# Autodesk Inventor assembly: main assembly
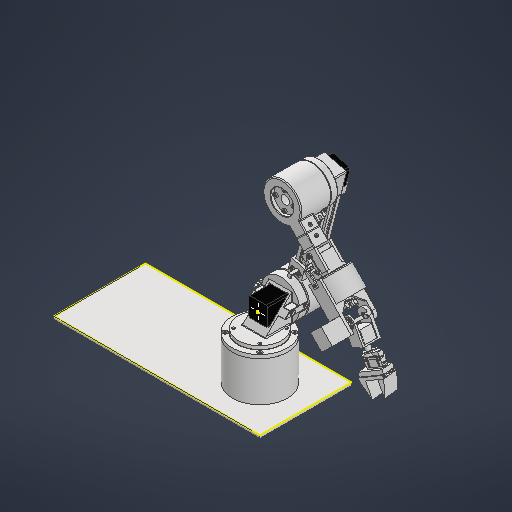
[picture p0: Inventor's stored thumbnail of the model, 512x512]
Saved by Autodesk Inventor 2026.1 (Build 301233020, 233B)
## iProperties
Created: 2025-07-04
Part Number: main assembly
Document SubType Name: Assembly
Designer: gavin
Author: gavin
## Documents named in this file (41)
- F:\temp data disk\Github\6-DOF-Robot-Arm\3D-model\robot armT 2(CAD file)\main assembly.iam
- F:\temp data disk\Github\6-DOF-Robot-Arm\3D-model\robot armT 2(CAD file)\stepper 42x48 - 27.ipt
- F:\temp data disk\Github\6-DOF-Robot-Arm\3D-model\robot armT 2(CAD file)\28stepper27.ipt
- F:\temp data disk\Github\6-DOF-Robot-Arm\3D-model\robot armT 2(CAD file)\CSN 02 4630 - 6009.ipt
- F:\temp data disk\Github\6-DOF-Robot-Arm\3D-model\robot armT 2(CAD file)\CNS 2862 B2116 - 6007 - 35 x 62 x 14.ipt
- F:\temp data disk\Github\6-DOF-Robot-Arm\3D-model\robot armT 2(CAD file)\base plate.ipt
- F:\temp data disk\Github\6-DOF-Robot-Arm\3D-model\robot armT 2(CAD file)\stepper 42x60 -50 .ipt
- F:\temp data disk\Github\6-DOF-Robot-Arm\3D-model\robot armT 2(CAD file)\j2 42 motor mount.ipt
- F:\temp data disk\Github\6-DOF-Robot-Arm\3D-model\robot armT 2(CAD file)\j1 assmble.iam
- F:\temp data disk\Github\6-DOF-Robot-Arm\3D-model\robot armT 2(CAD file)\optic endstop module.ipt
- F:\temp data disk\Github\6-DOF-Robot-Arm\3D-model\robot armT 2(CAD file)\j2j3 alumi ext.ipt
- F:\temp data disk\Github\6-DOF-Robot-Arm\3D-model\robot armT 2(CAD file)\j3 motor mount.ipt
- F:\temp data disk\Github\6-DOF-Robot-Arm\3D-model\robot armT 2(CAD file)\j3j4 alumi ext.ipt
- F:\temp data disk\Github\6-DOF-Robot-Arm\3D-model\robot armT 2(CAD file)\j2 endstop blocker.ipt
- F:\temp data disk\Github\6-DOF-Robot-Arm\3D-model\robot armT 2(CAD file)\j3 endstop blocker.ipt
- F:\temp data disk\Github\6-DOF-Robot-Arm\3D-model\robot armT 2(CAD file)\6mm axle hub.ipt
- F:\temp data disk\Github\6-DOF-Robot-Arm\3D-model\robot armT 2(CAD file)\j4 motor mount.ipt
- F:\temp data disk\Github\6-DOF-Robot-Arm\3D-model\robot armT 2(CAD file)\j4 motor mount cover.ipt
- F:\temp data disk\Github\6-DOF-Robot-Arm\3D-model\robot armT 2(CAD file)\j4 moving part.ipt
- F:\temp data disk\Github\6-DOF-Robot-Arm\3D-model\robot armT 2(CAD file)\nema 11x25.ipt
- F:\temp data disk\Github\6-DOF-Robot-Arm\3D-model\robot armT 2(CAD file)\5mm axle hub.ipt
- F:\temp data disk\Github\6-DOF-Robot-Arm\3D-model\robot armT 2(CAD file)\bearing 22-M6.ipt
- F:\temp data disk\Github\6-DOF-Robot-Arm\3D-model\robot armT 2(CAD file)\j6 motor mount v2.ipt
- F:\temp data disk\Github\6-DOF-Robot-Arm\3D-model\robot armT 2(CAD file)\j4 endstop blocker.ipt
- F:\temp data disk\Github\6-DOF-Robot-Arm\3D-model\robot armT 2(CAD file)\sg90 long claw.iam
- F:\temp data disk\Github\6-DOF-Robot-Arm\3D-model\robot armT 2(CAD file)\35x40 stepper.ipt
- F:\temp data disk\Github\6-DOF-Robot-Arm\3D-model\robot armT 2(CAD file)\j3 moving part option3.ipt
- F:\temp data disk\Github\6-DOF-Robot-Arm\3D-model\robot armT 2(CAD file)\z21 8x18.ipt
- F:\temp data disk\Github\6-DOF-Robot-Arm\3D-model\robot armT 2(CAD file)\18mm hub.ipt
- F:\temp data disk\Github\6-DOF-Robot-Arm\3D-model\robot armT 2(CAD file)\j2 moving part option2.ipt
- F:\temp data disk\Github\6-DOF-Robot-Arm\3D-model\robot armT 2(CAD file)\M5 heat set inserts.ipt
- F:\temp data disk\Github\6-DOF-Robot-Arm\3D-model\robot armT 2(CAD file)\AS 1427 - M3 x 6(5) II.ipt
- F:\temp data disk\Github\6-DOF-Robot-Arm\3D-model\robot armT 2(CAD file)\M3 heat set insert.ipt
- C:\Users\gavin\Documents\Inventor\Content Center Files\R2026\en-US\CNS 4557\CNS 4557 - M5 x 0.8 x 12.ipt
- F:\temp data disk\Github\6-DOF-Robot-Arm\3D-model\robot armT 2(CAD file)\CNS 4557 - M4 x 0.7 x 10.ipt
- F:\temp data disk\Github\6-DOF-Robot-Arm\3D-model\robot armT 2(CAD file)\AS 1474 - M4(1).ipt
- F:\temp data disk\Github\6-DOF-Robot-Arm\3D-model\robot armT 2(CAD file)\AS 1474 - M3(1).ipt
- C:\Users\gavin\Documents\Inventor\Content Center Files\R2026\en-US\AS 1112 (4)\AS 1112 - M6(2).ipt
- C:\Users\gavin\Documents\Inventor\Content Center Files\R2026\en-US\ASME ANSI B18.3.5M(2)\ASME_ANSI B18.3.5M - M3x6(2).ipt
- C:\Users\gavin\Documents\Inventor\Content Center Files\R2026\en-US\CNS 3932\CNS 3932 - M 4 x 0.7 x 10.ipt
- C:\Users\gavin\Documents\Inventor\Content Center Files\R2026\en-US\IS 7483\IS 7483 - M3 x 14.ipt
## Components (130 placed, 40 different names)
1. base plate:1 — Flush:5
2. j1 assmble:1 [sub-assembly]
3. stepper 42x48 - 27:2 — Mate:45, Mate:46, Mate:47, Mate:110, Flush:18
4. CSN 02 4630 - 6009:1 — Mate:48, Mate:49, Rotational:15
5. CSN 02 4630 - 6009:2 — Mate:16, Mate:29
6. CNS 2862 B2116 - 6007 - 35 x 62 x 14:1 — Mate:63, Mate:64, Rotational:16
7. stepper 42x60 -50 :1 — Mate:16, Mate:27, Mate:28, Mate:113, Flush:20
8. j2 42 motor mount:1 — Mate:27, Mate:28, Mate:29, Mate:33, Mate:34, Mate:35, Rigid:12, Rigid:13, Rigid:99, Rigid:100, Rigid:101, Rigid:102
9. optic endstop module:1 — Mate:33, Mate:34, Mate:35, Flush:10, Rigid:10, Rigid:11
10. j2j3 alumi ext:1 — Rigid:5, Rigid:7
11. j2j3 alumi ext:2 — Rigid:6
12. j3 motor mount:1 — Mate:45, Mate:46, Mate:47, Mate:48, Mate:49, Flush:11, Flush:12, Mate:59, Rigid:7, Mate:132, Rigid:65, Rigid:66, Rigid:67, Rigid:68, Rigid:95, Rigid:96, Rigid:97, Rigid:98
13. j3j4 alumi ext:1 — Rigid:4, Rigid:8
14. optic endstop module:2 — Mate:129, Mate:130, Mate:131, Rigid:20, Rigid:21, Rigid:22, Rigid:23
15. j2 endstop blocker:1 — Flush:10, Mate:117, Mate:118, Mate:119, Rigid:14, Rigid:15, Rigid:16, Rigid:17
16. j3 endstop blocker:1 — Flush:11, Flush:12, Mate:59, Mate:132, Rigid:18, Rigid:19, Rigid:24, Rigid:25
17. 6mm axle hub:1 — Mate:123, Mate:124, Mate:125
18. j4 motor mount:1 — Flush:14, Flush:15, Mate:62, Mate:63, Mate:65, Mate:71, Mate:72, Mate:73, Flush:21, Rigid:8, Rigid:9, Rigid:27, Rigid:28, Rigid:72, Rigid:75
19. j4 motor mount cover:1 — Flush:14, Flush:15, Mate:62, Mate:64, Mate:65
20. 28stepper27:1 — Rigid:9
21. optic endstop module:3 — Mate:71, Mate:72, Mate:73, Rigid:29, Rigid:30
22. j4 moving part:1 — Mate:74, Mate:76, Mate:86, Mate:87, Mate:104, Mate:105, Mate:107, Mate:108, Mate:109, Mate:123, Mate:124, Mate:125, Rotational:16, Mate:126, Mate:127, Rigid:26, Rigid:32, Rigid:33, Rigid:76, Rigid:77, Rigid:78, Rigid:79, Rigid:89, Rigid:90
23. nema 11x25:1 — Mate:88, Mate:89, Mate:102, Mate:103, Mate:128
24. optic endstop module:4 — Mate:74, Mate:76, Mate:107, Rigid:34, Rigid:35
25. 5mm axle hub:1 — Rigid:1, Rotational:12
26. bearing 22-M6:1 — Mate:86, Mate:87
27. j6 motor mount v2:1 — Mate:88, Mate:89, Rotational:12, Mate:128, Rigid:80, Rigid:81, Rigid:82, Rigid:83, Rigid:88
28. j4 endstop blocker:1 — Mate:108, Mate:109, Mate:126, Rigid:31
29. sg90 long claw:1 [sub-assembly] — Mate:99, Mate:100, Mate:101, Mate:103, Rigid:91, Rigid:92, Rigid:93, Rigid:94
30. 5mm axle hub:2 — Mate:99, Mate:100, Mate:101, Mate:102
31. 35x40 stepper:1 — Mate:104, Mate:105, Rigid:1, Mate:127
32. j3 moving part option3:1 — Rigid:4, Mate:120, Mate:121, Mate:122, Rotational:15, Flush:21, Mate:129, Mate:130, Mate:131, Rigid:40, Rigid:41, Rigid:42, Rigid:43, Rigid:73, Rigid:74
33. z21 8x18:1 — Mate:110, Flush:18
34. 18mm hub:1 — Mate:120, Mate:121, Mate:122, Rigid:44, Rigid:45, Rigid:46, Rigid:47
35. j2 moving part option2:1 — Rigid:5, Mate:114, Mate:115, Mate:116, Mate:117, Mate:118, Mate:119, Rigid:6, Rigid:36, Rigid:37, Rigid:38, Rigid:39, Rigid:59, Rigid:60, Rigid:61, Rigid:62
36. z21 8x18:2 — Rotational:14, Mate:113, Flush:20
37. 18mm hub:2 — Rotational:14, Mate:114, Mate:115, Mate:116, Rigid:48, Rigid:49, Rigid:50, Rigid:51
38. AS 1427 - M3 x 6(5) II:1 — Rigid:16
39. AS 1427 - M3 x 6(5) II:2 — Rigid:23
40. AS 1427 - M3 x 6(5) II:3 — Rigid:24
41. AS 1427 - M3 x 6(5) II:4 — Rigid:22
42. AS 1427 - M3 x 6(5) II:5 — Rigid:17
43. AS 1427 - M3 x 6(5) II:6 — Rigid:25
44. AS 1427 - M3 x 6(5) II:7 — Rigid:10
45. AS 1427 - M3 x 6(5) II:8 — Rigid:11
46. M3 heat set insert:1 — Rigid:15
47. M3 heat set insert:2 — Rigid:13
48. M3 heat set insert:3 — Rigid:26
49. M3 heat set insert:4 — Rigid:32
50. M3 heat set insert:5 — Rigid:28
51. M3 heat set insert:6 — Rigid:19
52. M3 heat set insert:7 — Rigid:20
53. M3 heat set insert:8 — Rigid:12
54. M3 heat set insert:9 — Rigid:14
55. M3 heat set insert:10 — Rigid:33
56. M3 heat set insert:14 — Rigid:27
57. M3 heat set insert:15 — Rigid:18
58. M3 heat set insert:18 — Rigid:21
59. AS 1427 - M3 x 6(5) II:9 — Rigid:29
60. AS 1427 - M3 x 6(5) II:10 — Rigid:35
61. AS 1427 - M3 x 6(5) II:11 — Rigid:31
62. AS 1427 - M3 x 6(5) II:12 — Rigid:30
63. AS 1427 - M3 x 6(5) II:13 — Rigid:34
64. M5 heat set inserts:5 — Rigid:39
65. M5 heat set inserts:6 — Rigid:36
66. M5 heat set inserts:10 — Rigid:42
67. M5 heat set inserts:11 — Rigid:41
68. M5 heat set inserts:12 — Rigid:40
69. M5 heat set inserts:13 — Rigid:38
70. M5 heat set inserts:14 — Rigid:37
71. M5 heat set inserts:18 — Rigid:43
72. CNS 4557 M5 x 12:1 — Rigid:45
73. CNS 4557 M5 x 12:2 — Rigid:44
74. CNS 4557 M5 x 12:3 — Rigid:49
75. CNS 4557 M5 x 12:4 — Rigid:48
76. CNS 4557 M5 x 12:5 — Rigid:47
77. CNS 4557 M5 x 12:6 — Rigid:46
78. CNS 4557 M5 x 12:7 — Rigid:51
79. CNS 4557 M5 x 12:8 — Rigid:50
80. CNS 4557 - M4 x 0.7 x 10:1 — Rigid:64, Rigid:65
81. CNS 4557 - M4 x 0.7 x 10:2 — Rigid:57, Rigid:60
82. CNS 4557 - M4 x 0.7 x 10:3 — Rigid:55, Rigid:74
83. CNS 4557 - M4 x 0.7 x 10:4 — Rigid:53, Rigid:67
84. CNS 4557 - M4 x 0.7 x 10:5 — Rigid:58, Rigid:59
85. CNS 4557 - M4 x 0.7 x 10:6 — Rigid:56, Rigid:62
86. CNS 4557 - M4 x 0.7 x 10:7 — Rigid:54, Rigid:68
87. CNS 4557 - M4 x 0.7 x 10:8 — Rigid:52, Rigid:61
88. CNS 4557 - M4 x 0.7 x 10:9 — Rigid:71, Rigid:72
89. CNS 4557 - M4 x 0.7 x 10:10 — Rigid:70, Rigid:73
90. CNS 4557 - M4 x 0.7 x 10:11 — Rigid:63, Rigid:66
91. CNS 4557 - M4 x 0.7 x 10:12 — Rigid:69, Rigid:75
92. AS 1474 - M4(1):1 — Rigid:57
93. AS 1474 - M4(1):2 — Rigid:55
94. AS 1474 - M4(1):3 — Rigid:92
95. AS 1474 - M4(1):4 — Rigid:91
96. AS 1474 - M4(1):5 — Rigid:56
97. AS 1474 - M4(1):6 — Rigid:53
98. AS 1474 - M4(1):7 — Rigid:54
99. AS 1474 - M4(1):11 — Rigid:64
100. AS 1474 - M4(1):12 — Rigid:63
101. AS 1474 - M4(1):13 — Rigid:71
102. AS 1474 - M4(1):14 — Rigid:69
103. AS 1474 - M4(1):15 — Rigid:70
104. AS 1474 - M4(1):16 — Rigid:52
105. AS 1474 - M4(1):18 — Rigid:58
106. AS 1474 - M3(1):1 — Rigid:87
107. AS 1474 - M3(1):2 — Rigid:86
108. AS 1474 - M3(1):3 — Rigid:84
109. AS 1474 - M3(1):5 — Rigid:85
110. AS 1112 (4) - Metric M6:1 — Rigid:88
111. Broached Hexagon Socket Flat Countersunk Head Cap Screws - Metric M3x6:1 — Rigid:77
112. Broached Hexagon Socket Flat Countersunk Head Cap Screws - Metric M3x6:2 — Rigid:78
113. Broached Hexagon Socket Flat Countersunk Head Cap Screws - Metric M3x6:3 — Rigid:80, Rigid:84
114. Broached Hexagon Socket Flat Countersunk Head Cap Screws - Metric M3x6:4 — Rigid:81, Rigid:85
115. Broached Hexagon Socket Flat Countersunk Head Cap Screws - Metric M3x6:5 — Rigid:76
116. Broached Hexagon Socket Flat Countersunk Head Cap Screws - Metric M3x6:6 — Rigid:79
117. CNS 3932 M 4 x 10:1 — Rigid:89
118. CNS 3932 M 4 x 10:4 — Rigid:90
119. IS 7483 M3 x 14:1 — Rigid:93
120. IS 7483 M3 x 14:2 — Rigid:94
121. Broached Hexagon Socket Flat Countersunk Head Cap Screws - Metric M3x6:7 — Rigid:83, Rigid:87
122. Broached Hexagon Socket Flat Countersunk Head Cap Screws - Metric M3x6:8 — Rigid:82, Rigid:86
123. Broached Hexagon Socket Flat Countersunk Head Cap Screws - Metric M3x6:9 — Rigid:97
124. Broached Hexagon Socket Flat Countersunk Head Cap Screws - Metric M3x6:10 — Rigid:95
125. Broached Hexagon Socket Flat Countersunk Head Cap Screws - Metric M3x6:11 — Rigid:99
126. Broached Hexagon Socket Flat Countersunk Head Cap Screws - Metric M3x6:12 — Rigid:101
127. Broached Hexagon Socket Flat Countersunk Head Cap Screws - Metric M3x6:13 — Rigid:96
128. Broached Hexagon Socket Flat Countersunk Head Cap Screws - Metric M3x6:14 — Rigid:98
129. Broached Hexagon Socket Flat Countersunk Head Cap Screws - Metric M3x6:15 — Rigid:100
130. Broached Hexagon Socket Flat Countersunk Head Cap Screws - Metric M3x6:16 — Rigid:102
## Relationships (184: WeldJoint 100, Mate 64, Flush 10, RevoluteJoint 10)
- [Mate]: j1 assmble:1
- [Flush]: base plate:1 ↔ j1 assmble:1
- [Mate]: base plate:1 ↔ j1 assmble:1
- Flush:5: base plate:1
- Mate:16: CSN 02 4630 - 6009:2 ↔ stepper 42x60 -50 :1
- [Mate] (20 mm): j1 assmble:1 ↔ stepper 42x60 -50 :1
- [Mate]: j1 assmble:1 ↔ j2 42 motor mount:1
- [Mate]: base plate:1 ↔ j1 assmble:1
- [Mate]: j1 assmble:1 ↔ j2 42 motor mount:1
- [Mate]: j1 assmble:1 ↔ j2 42 motor mount:1
- Mate:27: stepper 42x60 -50 :1 ↔ j2 42 motor mount:1
- Mate:28: stepper 42x60 -50 :1 ↔ j2 42 motor mount:1
- Mate:29: CSN 02 4630 - 6009:2 ↔ j2 42 motor mount:1
- [RevoluteJoint]: base plate:1 ↔ j1 assmble:1
- [RevoluteJoint]: base plate:1 ↔ j1 assmble:1
- [RevoluteJoint]: base plate:1 ↔ j1 assmble:1
- [RevoluteJoint]: base plate:1 ↔ j1 assmble:1
- [RevoluteJoint]: base plate:1 ↔ j1 assmble:1
- [RevoluteJoint]: base plate:1 ↔ j1 assmble:1
- Mate:33: j2 42 motor mount:1 ↔ optic endstop module:1
- Mate:34: j2 42 motor mount:1 ↔ optic endstop module:1
- Mate:35: j2 42 motor mount:1 ↔ optic endstop module:1
- Mate:45: stepper 42x48 - 27:2 ↔ j3 motor mount:1
- Mate:46 (0.075 mm): stepper 42x48 - 27:2 ↔ j3 motor mount:1
- Mate:47: stepper 42x48 - 27:2 ↔ j3 motor mount:1
- Mate:48: CSN 02 4630 - 6009:1 ↔ j3 motor mount:1
- Mate:49: CSN 02 4630 - 6009:1 ↔ j3 motor mount:1
- Flush:10: optic endstop module:1 ↔ j2 endstop blocker:1
- Flush:11: j3 motor mount:1 ↔ j3 endstop blocker:1
- Flush:12: j3 motor mount:1 ↔ j3 endstop blocker:1
- Flush:14: j4 motor mount:1 ↔ j4 motor mount cover:1
- Flush:15: j4 motor mount:1 ↔ j4 motor mount cover:1
- Mate:59: j3 motor mount:1 ↔ j3 endstop blocker:1
- Mate:62: j4 motor mount:1 ↔ j4 motor mount cover:1
- Mate:63: CNS 2862 B2116 - 6007 - 35 x 62 x 14:1 ↔ j4 motor mount:1
- Mate:64: CNS 2862 B2116 - 6007 - 35 x 62 x 14:1 ↔ j4 motor mount cover:1
- Mate:65: j4 motor mount:1 ↔ j4 motor mount cover:1
- Mate:71: j4 motor mount:1 ↔ optic endstop module:3
- Mate:72: j4 motor mount:1 ↔ optic endstop module:3
- Mate:73: j4 motor mount:1 ↔ optic endstop module:3
- Mate:74: j4 moving part:1 ↔ optic endstop module:4
- Mate:76: j4 moving part:1 ↔ optic endstop module:4
- Mate:86: j4 moving part:1 ↔ bearing 22-M6:1
- Mate:87: j4 moving part:1 ↔ bearing 22-M6:1
- Mate:88: nema 11x25:1 ↔ j6 motor mount v2:1
- Mate:89: nema 11x25:1 ↔ j6 motor mount v2:1
- Mate:99: sg90 long claw:1 ↔ 5mm axle hub:2
- Mate:100: sg90 long claw:1 ↔ 5mm axle hub:2
- Mate:101: sg90 long claw:1 ↔ 5mm axle hub:2
- Mate:102: nema 11x25:1 ↔ 5mm axle hub:2
- Mate:103: nema 11x25:1 ↔ sg90 long claw:1
- Mate:104: j4 moving part:1 ↔ 35x40 stepper:1
- Mate:105: j4 moving part:1 ↔ 35x40 stepper:1
- Rigid:1 [WeldJoint]: 5mm axle hub:1 ↔ 35x40 stepper:1
- Rotational:12 [RevoluteJoint]: 5mm axle hub:1 ↔ j6 motor mount v2:1
- Mate:107: j4 moving part:1 ↔ optic endstop module:4
- Mate:108: j4 moving part:1 ↔ j4 endstop blocker:1
- Mate:109: j4 moving part:1 ↔ j4 endstop blocker:1
- Mate:110: stepper 42x48 - 27:2 ↔ z21 8x18:1
- Flush:18: stepper 42x48 - 27:2 ↔ z21 8x18:1
- Rotational:14 [RevoluteJoint] (-3.71 mm): z21 8x18:2 ↔ 18mm hub:2
- Mate:113: stepper 42x60 -50 :1 ↔ z21 8x18:2
- Flush:20: stepper 42x60 -50 :1 ↔ z21 8x18:2
- Rigid:4 [WeldJoint]: j3j4 alumi ext:1 ↔ j3 moving part option3:1
- Rigid:5 [WeldJoint]: j2j3 alumi ext:1 ↔ j2 moving part option2:1
- Mate:114: j2 moving part option2:1 ↔ 18mm hub:2
- Mate:115: j2 moving part option2:1 ↔ 18mm hub:2
- Mate:116: j2 moving part option2:1 ↔ 18mm hub:2
- Mate:117: j2 endstop blocker:1 ↔ j2 moving part option2:1
- Mate:118: j2 endstop blocker:1 ↔ j2 moving part option2:1
- Mate:119: j2 endstop blocker:1 ↔ j2 moving part option2:1
- Rigid:6 [WeldJoint]: j2j3 alumi ext:2 ↔ j2 moving part option2:1
- Rigid:7 [WeldJoint]: j2j3 alumi ext:1 ↔ j3 motor mount:1
- Mate:120: j3 moving part option3:1 ↔ 18mm hub:1
- Mate:121: j3 moving part option3:1 ↔ 18mm hub:1
- Mate:122: j3 moving part option3:1 ↔ 18mm hub:1
- Rotational:15 [RevoluteJoint]: CSN 02 4630 - 6009:1 ↔ j3 moving part option3:1
- Flush:21: j4 motor mount:1 ↔ j3 moving part option3:1
- Rigid:8 [WeldJoint]: j3j4 alumi ext:1 ↔ j4 motor mount:1
- Rigid:9 [WeldJoint]: j4 motor mount:1 ↔ 28stepper27:1
- Mate:123: 6mm axle hub:1 ↔ j4 moving part:1
- Mate:124: 6mm axle hub:1 ↔ j4 moving part:1
- Mate:125: 6mm axle hub:1 ↔ j4 moving part:1
- Rotational:16 [RevoluteJoint]: CNS 2862 B2116 - 6007 - 35 x 62 x 14:1 ↔ j4 moving part:1
- Mate:126: j4 moving part:1 ↔ j4 endstop blocker:1
- Mate:127: j4 moving part:1 ↔ 35x40 stepper:1
- Mate:128: nema 11x25:1 ↔ j6 motor mount v2:1
- Mate:129: optic endstop module:2 ↔ j3 moving part option3:1
- Mate:130: optic endstop module:2 ↔ j3 moving part option3:1
- Mate:131: optic endstop module:2 ↔ j3 moving part option3:1
- Mate:132: j3 motor mount:1 ↔ j3 endstop blocker:1
- Rigid:10 [WeldJoint]: optic endstop module:1 ↔ AS 1427 - M3 x 6(5) II:7
- Rigid:11 [WeldJoint]: optic endstop module:1 ↔ AS 1427 - M3 x 6(5) II:8
- Rigid:12 [WeldJoint]: j2 42 motor mount:1 ↔ M3 heat set insert:8
- Rigid:13 [WeldJoint]: j2 42 motor mount:1 ↔ M3 heat set insert:2
- Rigid:14 [WeldJoint]: j2 endstop blocker:1 ↔ M3 heat set insert:9
- Rigid:15 [WeldJoint]: j2 endstop blocker:1 ↔ M3 heat set insert:1
- Rigid:16 [WeldJoint]: j2 endstop blocker:1 ↔ AS 1427 - M3 x 6(5) II:1
- Rigid:17 [WeldJoint]: j2 endstop blocker:1 ↔ AS 1427 - M3 x 6(5) II:5
- Rigid:18 [WeldJoint]: j3 endstop blocker:1 ↔ M3 heat set insert:15
- Rigid:19 [WeldJoint]: j3 endstop blocker:1 ↔ M3 heat set insert:6
- Rigid:20 [WeldJoint]: optic endstop module:2 ↔ M3 heat set insert:7
- Rigid:21 [WeldJoint]: optic endstop module:2 ↔ M3 heat set insert:18
- Rigid:22 [WeldJoint]: optic endstop module:2 ↔ AS 1427 - M3 x 6(5) II:4
- Rigid:23 [WeldJoint]: optic endstop module:2 ↔ AS 1427 - M3 x 6(5) II:2
- Rigid:24 [WeldJoint]: j3 endstop blocker:1 ↔ AS 1427 - M3 x 6(5) II:3
- Rigid:25 [WeldJoint]: j3 endstop blocker:1 ↔ AS 1427 - M3 x 6(5) II:6
- Rigid:26 [WeldJoint]: j4 moving part:1 ↔ M3 heat set insert:3
- Rigid:27 [WeldJoint]: j4 motor mount:1 ↔ M3 heat set insert:14
- Rigid:28 [WeldJoint]: j4 motor mount:1 ↔ M3 heat set insert:5
- Rigid:29 [WeldJoint]: optic endstop module:3 ↔ AS 1427 - M3 x 6(5) II:9
- Rigid:30 [WeldJoint]: optic endstop module:3 ↔ AS 1427 - M3 x 6(5) II:12
- Rigid:31 [WeldJoint]: j4 endstop blocker:1 ↔ AS 1427 - M3 x 6(5) II:11
- Rigid:32 [WeldJoint]: j4 moving part:1 ↔ M3 heat set insert:4
- Rigid:33 [WeldJoint]: j4 moving part:1 ↔ M3 heat set insert:10
- Rigid:34 [WeldJoint]: optic endstop module:4 ↔ AS 1427 - M3 x 6(5) II:13
- Rigid:35 [WeldJoint]: optic endstop module:4 ↔ AS 1427 - M3 x 6(5) II:10
- Rigid:36 [WeldJoint]: j2 moving part option2:1 ↔ M5 heat set inserts:6
- Rigid:37 [WeldJoint]: j2 moving part option2:1 ↔ M5 heat set inserts:14
- Rigid:38 [WeldJoint]: j2 moving part option2:1 ↔ M5 heat set inserts:13
- Rigid:39 [WeldJoint]: j2 moving part option2:1 ↔ M5 heat set inserts:5
- Rigid:40 [WeldJoint]: j3 moving part option3:1 ↔ M5 heat set inserts:12
- Rigid:41 [WeldJoint]: j3 moving part option3:1 ↔ M5 heat set inserts:11
- Rigid:42 [WeldJoint]: j3 moving part option3:1 ↔ M5 heat set inserts:10
- Rigid:43 [WeldJoint]: j3 moving part option3:1 ↔ M5 heat set inserts:18
- Rigid:44 [WeldJoint]: 18mm hub:1 ↔ CNS 4557 M5 x 12:2
- Rigid:45 [WeldJoint]: 18mm hub:1 ↔ CNS 4557 M5 x 12:1
- Rigid:46 [WeldJoint]: 18mm hub:1 ↔ CNS 4557 M5 x 12:6
- Rigid:47 [WeldJoint]: 18mm hub:1 ↔ CNS 4557 M5 x 12:5
- Rigid:48 [WeldJoint]: 18mm hub:2 ↔ CNS 4557 M5 x 12:4
- Rigid:49 [WeldJoint]: 18mm hub:2 ↔ CNS 4557 M5 x 12:3
- Rigid:50 [WeldJoint]: 18mm hub:2 ↔ CNS 4557 M5 x 12:8
- Rigid:51 [WeldJoint]: 18mm hub:2 ↔ CNS 4557 M5 x 12:7
- Rigid:52 [WeldJoint] (10 mm): CNS 4557 - M4 x 0.7 x 10:8 ↔ AS 1474 - M4(1):16
- Rigid:53 [WeldJoint]: CNS 4557 - M4 x 0.7 x 10:4 ↔ AS 1474 - M4(1):6
- Rigid:54 [WeldJoint]: CNS 4557 - M4 x 0.7 x 10:7 ↔ AS 1474 - M4(1):7
- Rigid:55 [WeldJoint]: CNS 4557 - M4 x 0.7 x 10:3 ↔ AS 1474 - M4(1):2
- Rigid:56 [WeldJoint]: CNS 4557 - M4 x 0.7 x 10:6 ↔ AS 1474 - M4(1):5
- Rigid:57 [WeldJoint]: CNS 4557 - M4 x 0.7 x 10:2 ↔ AS 1474 - M4(1):1
- Rigid:58 [WeldJoint]: CNS 4557 - M4 x 0.7 x 10:5 ↔ AS 1474 - M4(1):18
- Rigid:59 [WeldJoint]: j2 moving part option2:1 ↔ CNS 4557 - M4 x 0.7 x 10:5
- Rigid:60 [WeldJoint]: j2 moving part option2:1 ↔ CNS 4557 - M4 x 0.7 x 10:2
- Rigid:61 [WeldJoint]: j2 moving part option2:1 ↔ CNS 4557 - M4 x 0.7 x 10:8
- Rigid:62 [WeldJoint]: j2 moving part option2:1 ↔ CNS 4557 - M4 x 0.7 x 10:6
- Rigid:63 [WeldJoint]: CNS 4557 - M4 x 0.7 x 10:11 ↔ AS 1474 - M4(1):12
- Rigid:64 [WeldJoint]: CNS 4557 - M4 x 0.7 x 10:1 ↔ AS 1474 - M4(1):11
- Rigid:65 [WeldJoint]: j3 motor mount:1 ↔ CNS 4557 - M4 x 0.7 x 10:1
- Rigid:66 [WeldJoint]: j3 motor mount:1 ↔ CNS 4557 - M4 x 0.7 x 10:11
- Rigid:67 [WeldJoint]: j3 motor mount:1 ↔ CNS 4557 - M4 x 0.7 x 10:4
- Rigid:68 [WeldJoint]: j3 motor mount:1 ↔ CNS 4557 - M4 x 0.7 x 10:7
- Rigid:69 [WeldJoint]: CNS 4557 - M4 x 0.7 x 10:12 ↔ AS 1474 - M4(1):14
- Rigid:70 [WeldJoint]: CNS 4557 - M4 x 0.7 x 10:10 ↔ AS 1474 - M4(1):15
- Rigid:71 [WeldJoint]: CNS 4557 - M4 x 0.7 x 10:9 ↔ AS 1474 - M4(1):13
- Rigid:72 [WeldJoint]: j4 motor mount:1 ↔ CNS 4557 - M4 x 0.7 x 10:9
- Rigid:73 [WeldJoint]: j3 moving part option3:1 ↔ CNS 4557 - M4 x 0.7 x 10:10
- Rigid:74 [WeldJoint]: j3 moving part option3:1 ↔ CNS 4557 - M4 x 0.7 x 10:3
- Rigid:75 [WeldJoint]: j4 motor mount:1 ↔ CNS 4557 - M4 x 0.7 x 10:12
- Rigid:76 [WeldJoint]: j4 moving part:1 ↔ Broached Hexagon Socket Flat Countersunk Head Cap Screws - Metric M3x6:5
- Rigid:77 [WeldJoint]: j4 moving part:1 ↔ Broached Hexagon Socket Flat Countersunk Head Cap Screws - Metric M3x6:1
- Rigid:78 [WeldJoint]: j4 moving part:1 ↔ Broached Hexagon Socket Flat Countersunk Head Cap Screws - Metric M3x6:2
- Rigid:79 [WeldJoint]: j4 moving part:1 ↔ Broached Hexagon Socket Flat Countersunk Head Cap Screws - Metric M3x6:6
- Rigid:80 [WeldJoint]: j6 motor mount v2:1 ↔ Broached Hexagon Socket Flat Countersunk Head Cap Screws - Metric M3x6:3
- Rigid:81 [WeldJoint]: j6 motor mount v2:1 ↔ Broached Hexagon Socket Flat Countersunk Head Cap Screws - Metric M3x6:4
- Rigid:82 [WeldJoint]: j6 motor mount v2:1 ↔ Broached Hexagon Socket Flat Countersunk Head Cap Screws - Metric M3x6:8
- Rigid:83 [WeldJoint]: j6 motor mount v2:1 ↔ Broached Hexagon Socket Flat Countersunk Head Cap Screws - Metric M3x6:7
- Rigid:84 [WeldJoint]: AS 1474 - M3(1):3 ↔ Broached Hexagon Socket Flat Countersunk Head Cap Screws - Metric M3x6:3
- Rigid:85 [WeldJoint]: AS 1474 - M3(1):5 ↔ Broached Hexagon Socket Flat Countersunk Head Cap Screws - Metric M3x6:4
- Rigid:86 [WeldJoint]: AS 1474 - M3(1):2 ↔ Broached Hexagon Socket Flat Countersunk Head Cap Screws - Metric M3x6:8
- Rigid:87 [WeldJoint]: AS 1474 - M3(1):1 ↔ Broached Hexagon Socket Flat Countersunk Head Cap Screws - Metric M3x6:7
- Rigid:88 [WeldJoint]: j6 motor mount v2:1 ↔ AS 1112 (4) - Metric M6:1
- Rigid:89 [WeldJoint]: j4 moving part:1 ↔ CNS 3932 M 4 x 10:1
- Rigid:90 [WeldJoint]: j4 moving part:1 ↔ CNS 3932 M 4 x 10:4
- Rigid:91 [WeldJoint]: sg90 long claw:1 ↔ AS 1474 - M4(1):4
- Rigid:92 [WeldJoint]: sg90 long claw:1 ↔ AS 1474 - M4(1):3
- Rigid:93 [WeldJoint]: sg90 long claw:1 ↔ IS 7483 M3 x 14:1
- Rigid:94 [WeldJoint]: sg90 long claw:1 ↔ IS 7483 M3 x 14:2
- Rigid:95 [WeldJoint]: j3 motor mount:1 ↔ Broached Hexagon Socket Flat Countersunk Head Cap Screws - Metric M3x6:10
- Rigid:96 [WeldJoint]: j3 motor mount:1 ↔ Broached Hexagon Socket Flat Countersunk Head Cap Screws - Metric M3x6:13
- Rigid:97 [WeldJoint]: j3 motor mount:1 ↔ Broached Hexagon Socket Flat Countersunk Head Cap Screws - Metric M3x6:9
- Rigid:98 [WeldJoint]: j3 motor mount:1 ↔ Broached Hexagon Socket Flat Countersunk Head Cap Screws - Metric M3x6:14
- Rigid:99 [WeldJoint]: j2 42 motor mount:1 ↔ Broached Hexagon Socket Flat Countersunk Head Cap Screws - Metric M3x6:11
- Rigid:100 [WeldJoint]: j2 42 motor mount:1 ↔ Broached Hexagon Socket Flat Countersunk Head Cap Screws - Metric M3x6:15
- Rigid:101 [WeldJoint]: j2 42 motor mount:1 ↔ Broached Hexagon Socket Flat Countersunk Head Cap Screws - Metric M3x6:12
- Rigid:102 [WeldJoint]: j2 42 motor mount:1 ↔ Broached Hexagon Socket Flat Countersunk Head Cap Screws - Metric M3x6:16
## Named parameters: d225_d219 = -3.71 mm
